# Autodesk Inventor assembly: Gripper Assembly
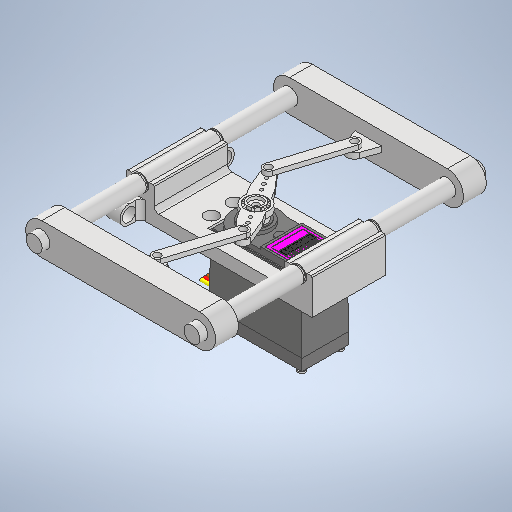
[picture p0: Inventor's stored thumbnail of the model, 512x512]
Saved by Autodesk Inventor 2025.2 (Build 292293000, 293)
## iProperties
Created: 2025-01-12
Part Number: Gripper Assembly
Document SubType Name: Assembly
Designer: caomi
Author: caomi
## Documents named in this file (7)
- C:\Minh Nguyen\H2A\cad\Gripper\Gripper Assembly.iam
- C:\Minh Nguyen\H2A\cad\Gripper\mg996R_v2\mg996R_v2\mg996R_v2.ipt
- C:\Minh Nguyen\H2A\cad\Gripper\Servo mount - front.ipt
- C:\Minh Nguyen\H2A\cad\Gripper\Linear Rod.ipt
- C:\Minh Nguyen\H2A\cad\Gripper\Gripper_arms.ipt
- C:\Minh Nguyen\H2A\cad\Gripper\Servo connector.ipt
- C:\Minh Nguyen\H2A\cad\Gripper\Servo horn.ipt
## Components (9 placed, 6 different names)
1. mg996R_v2:1 — Rigid:1, Rotational:2
2. Servo mount - front:1 — Rigid:1, Rigid:2, Rigid:3
3. Linear Rod:1 — Rigid:2, Cylindrical:1, Cylindrical:3
4. Linear Rod:2 — Rigid:3, Cylindrical:2, Cylindrical:4
5. Gripper_arms:1 — Cylindrical:1, Cylindrical:2, Rotational:1
6. Gripper_arms:2 — Cylindrical:3, Cylindrical:4, Rotational:3
7. Servo connector:1 — Rotational:1, Cylindrical:5
8. Servo horn:1 — Rotational:2, Cylindrical:5, Cylindrical:6
9. Servo connector:2 — Rotational:3, Cylindrical:6
## Relationships (12: CylindricalJoint 6, WeldJoint 3, RevoluteJoint 3)
- Rigid:1 [WeldJoint]: mg996R_v2:1 ↔ Servo mount - front:1
- Rigid:2 [WeldJoint]: Servo mount - front:1 ↔ Linear Rod:1
- Rigid:3 [WeldJoint]: Servo mount - front:1 ↔ Linear Rod:2
- Cylindrical:1: Linear Rod:1 ↔ Gripper_arms:1
- Cylindrical:2: Linear Rod:2 ↔ Gripper_arms:1
- Cylindrical:3: Linear Rod:1 ↔ Gripper_arms:2
- Cylindrical:4: Linear Rod:2 ↔ Gripper_arms:2
- Rotational:1 [RevoluteJoint]: Gripper_arms:1 ↔ Servo connector:1
- Rotational:2 [RevoluteJoint]: mg996R_v2:1 ↔ Servo horn:1
- Cylindrical:5: Servo connector:1 ↔ Servo horn:1
- Rotational:3 [RevoluteJoint]: Gripper_arms:2 ↔ Servo connector:2
- Cylindrical:6: Servo horn:1 ↔ Servo connector:2
